# Autodesk Inventor assembly: Gripper1
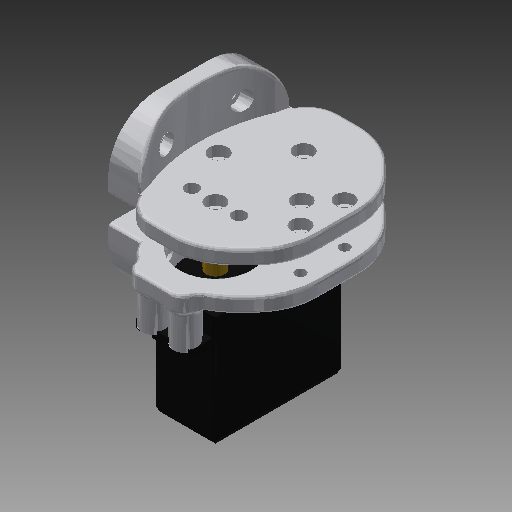
[picture p0: Inventor's stored thumbnail of the model, 512x512]
Saved by Autodesk Inventor 2017 SP1 (Build 210196100, 196)
## iProperties
Created: 2018-03-03
Part Number: Gripper1
Document SubType Name: Assembly
Designer: Zach
Author: Zach
## Documents named in this file (2)
- C:\Users\Zach\Documents\GitHub\tr1_description\meshes\Visual Assembly\Gripper1.iam
- C:\Users\Zach\Documents\GitHub\tr1_description\meshes\Visual Assembly\Gripper1.ipt
## Components (1 placed, 1 different names)
1. Gripper1:1 — Mate:1, Flush:1, Mate:2, Mate:3
## Relationships (4: Mate 3, Flush 1)
- Mate:1: Gripper1:1
- Flush:1 (-4 mm): Gripper1:1
- Mate:2: Gripper1:1
- Mate:3: Gripper1:1
